# Autodesk Inventor assembly: activeMarker
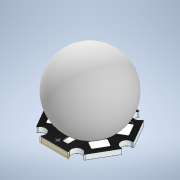
[picture p0: Inventor's stored thumbnail of the model, 180x180]
Saved by Autodesk Inventor 2022 (Build 260153000, 153)
## iProperties
Created: 2021-09-02
Part Number: activeMarker
Document SubType Name: Assembly
Designer: tecware
Author: tecware
## Documents named in this file (4)
- C:\Users\tecware\Documents\Inventor\activeMarker\activeMarker.iam
- C:\Users\tecware\Documents\newCamera\cad\star-lambertian-3w-led.snapshot.3\Star-Lambertian-1\Star-Lambertian-1.iam
- C:\Users\tecware\Documents\Inventor\activeMarker\marker.ipt
- C:\Users\tecware\Documents\Inventor\activeMarker\markerHalf.ipt
## Components (3 placed, 3 different names)
1. Star-Lambertian-1:1 [sub-assembly] — Flush:1, Flush:2, Mate:1, Mate:2
2. marker:1 — Flush:1
3. markerHalf:1 — Flush:2, Mate:1, Mate:2
## Relationships (4: Flush 2, Mate 2)
- Flush:1: Star-Lambertian-1:1 ↔ marker:1
- Flush:2: Star-Lambertian-1:1 ↔ markerHalf:1
- Mate:1: Star-Lambertian-1:1 ↔ markerHalf:1
- Mate:2: Star-Lambertian-1:1 ↔ markerHalf:1
